# Autodesk Inventor assembly: Perna_Esq_Montada_v1
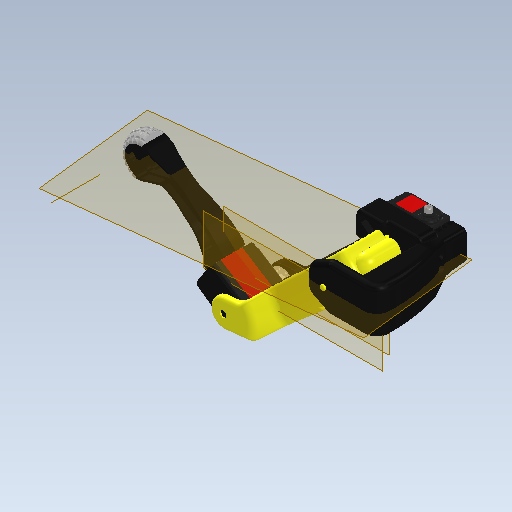
[picture p0: Inventor's stored thumbnail of the model, 512x512]
Saved by Autodesk Inventor 2020 (Build 240168000, 168)
## iProperties
Created: 2021-05-13
Part Number: Perna_Esq_Montada_v1
Document SubType Name: Assembly
Designer: JCarlos
Author: JCarlos
## Documents named in this file (10)
- C:\Users\candu\Google Drive\Doutorado_UTFPR\Projeto_1_SpotMicro\Projeto_3D\Robo_Montado_v3\Perna_Esq_Montada_v3.iam
- C:\Users\candu\Google Drive\Doutorado_UTFPR\Projeto_1_SpotMicro\Projeto_3D\Robo_Montado_v3\Braço_Esq.ipt
- C:\Users\candu\Google Drive\Doutorado_UTFPR\Projeto_1_SpotMicro\Projeto_3D\Robo_Montado_v3\Ante_Braço_Esq.ipt
- C:\Users\candu\Google Drive\Doutorado_UTFPR\Projeto_1_SpotMicro\Projeto_3D\Perna_Esq_Montada_v1\Design Accelerator\Rolamento1.iam
- C:\Users\candu\Google Drive\Doutorado_UTFPR\Projeto_1_SpotMicro\Projeto_3D\Robo_Montado_v3\foot.ipt
- C:\Users\candu\Google Drive\Doutorado_UTFPR\Projeto_1_SpotMicro\Projeto_3D\Robo_Montado_v3\Cover_Braço_Esq_v3.ipt
- C:\Users\candu\Google Drive\Doutorado_UTFPR\Projeto_1_SpotMicro\Projeto_3D\Robo_Montado_v3\LF20MG\Circle Rudder.ipt
- C:\Users\candu\Google Drive\Doutorado_UTFPR\Projeto_1_SpotMicro\Projeto_3D\Robo_Montado_v3\LF20MG\LF20MG.ipt
- C:\Users\candu\Google Drive\Doutorado_UTFPR\Projeto_1_SpotMicro\Projeto_3D\Robo_Montado_v3\Rótula_FrEsq_TrDir_v3.ipt
- C:\Users\candu\Google Drive\Doutorado_UTFPR\Projeto_1_SpotMicro\Projeto_3D\Robo_Montado_v3\Ombrera_Esq.ipt
## Components (11 placed, 9 different names)
1. LF20MG:3 — Coincidência:46, Coincidência:47, Coincidência:48, Coincidência:49, Coincidência:50
2. Braço_Esq:1 — Coincidência:8, Alinhamento:3, Coincidência:44, Coincidência:45, Coincidência:46, Coincidência:47, Coincidência:48, Coincidência:62, Tangente:2
3. Ante_Braço_Esq:1 — Coincidência:5, Alinhamento:1, Coincidência:7, Simetria:1, Coincidência:34, Coincidência:36, Coincidência:43, Coincidência:51, Coincidência:52, Coincidência:53
4. Cover_Braço_Esq_v3:1 — Coincidência:5, Alinhamento:1, Coincidência:7, Coincidência:8, Ângulo:1, Tangente:1, Coincidência:33, Alinhamento:2, Coincidência:64, Coincidência:65
5. Rolamento:1 [sub-assembly] — Coincidência:33, Alinhamento:2
6. LF20MG:2 — Coincidência:51, Coincidência:52, Coincidência:53, Coincidência:54, Coincidência:55
7. Circle Rudder:1 — Coincidência:34, Coincidência:36, Coincidência:43, Coincidência:49, Coincidência:50
8. foot:1 — Alinhamento:3, Coincidência:44, Coincidência:45
9. Rótula_FrEsq_TrDir_v3:1 — Coincidência:54, Coincidência:55, Ângulo:2, Coincidência:56, Coincidência:57, Coincidência:58, Ângulo:3, Alinhamento:4
10. LF20MG:4 — Coincidência:56, Coincidência:57, Coincidência:58, Coincidência:59, Coincidência:60, Coincidência:61
11. Ombrera_Esq:1 — Coincidência:59, Coincidência:60, Coincidência:61
## Relationships (39: Mate 29, Flush 4, Angle 3, Tangent 2, Symmetry 1)
- Coincidência:5 [Mate]: Ante_Braço_Esq:1 ↔ Cover_Braço_Esq_v3:1
- Alinhamento:1 [Flush]: Ante_Braço_Esq:1 ↔ Cover_Braço_Esq_v3:1
- Coincidência:7 [Mate]: Ante_Braço_Esq:1 ↔ Cover_Braço_Esq_v3:1
- Coincidência:8 [Mate] (1 mm): Braço_Esq:1 ↔ Cover_Braço_Esq_v3:1
- Ângulo:1 [Angle] (0 deg): Cover_Braço_Esq_v3:1
- Tangente:1: Cover_Braço_Esq_v3:1
- Simetria:1 [Symmetry]: Ante_Braço_Esq:1
- Coincidência:33 [Mate]: Cover_Braço_Esq_v3:1 ↔ Rolamento:1
- Alinhamento:2 [Flush]: Cover_Braço_Esq_v3:1 ↔ Rolamento:1
- Coincidência:34 [Mate]: Ante_Braço_Esq:1 ↔ Circle Rudder:1
- Coincidência:36 [Mate]: Ante_Braço_Esq:1 ↔ Circle Rudder:1
- Coincidência:43 [Mate]: Ante_Braço_Esq:1 ↔ Circle Rudder:1
- Alinhamento:3 [Flush]: Braço_Esq:1 ↔ foot:1
- Coincidência:44 [Mate]: Braço_Esq:1 ↔ foot:1
- Coincidência:45 [Mate]: Braço_Esq:1 ↔ foot:1
- Coincidência:46 [Mate]: LF20MG:3 ↔ Braço_Esq:1
- Coincidência:47 [Mate]: LF20MG:3 ↔ Braço_Esq:1
- Coincidência:48 [Mate]: LF20MG:3 ↔ Braço_Esq:1
- Coincidência:49 [Mate] (-46 mm): LF20MG:3 ↔ Circle Rudder:1
- Coincidência:50 [Mate]: LF20MG:3 ↔ Circle Rudder:1
- Coincidência:51 [Mate]: Ante_Braço_Esq:1 ↔ LF20MG:2
- Coincidência:52 [Mate]: Ante_Braço_Esq:1 ↔ LF20MG:2
- Coincidência:53 [Mate]: Ante_Braço_Esq:1 ↔ LF20MG:2
- Coincidência:54 [Mate]: LF20MG:2 ↔ Rótula_FrEsq_TrDir_v3:1
- Coincidência:55 [Mate] (3 mm): LF20MG:2 ↔ Rótula_FrEsq_TrDir_v3:1
- Ângulo:2 [Angle] (90 deg): Rótula_FrEsq_TrDir_v3:1
- Coincidência:56 [Mate]: Rótula_FrEsq_TrDir_v3:1 ↔ LF20MG:4
- Coincidência:57 [Mate]: Rótula_FrEsq_TrDir_v3:1 ↔ LF20MG:4
- Coincidência:58 [Mate]: Rótula_FrEsq_TrDir_v3:1 ↔ LF20MG:4
- Coincidência:59 [Mate]: LF20MG:4 ↔ Ombrera_Esq:1
- Coincidência:60 [Mate]: LF20MG:4 ↔ Ombrera_Esq:1
- Coincidência:61 [Mate] (0.5 mm): LF20MG:4 ↔ Ombrera_Esq:1
- Coincidência:62 [Mate]: Braço_Esq:1
- Coincidência:63 [Mate]
- Ângulo:3 [Angle] (90 deg): Rótula_FrEsq_TrDir_v3:1
- Tangente:2: Braço_Esq:1
- Alinhamento:4 [Flush]: Rótula_FrEsq_TrDir_v3:1
- Coincidência:64 [Mate]: Cover_Braço_Esq_v3:1
- Coincidência:65 [Mate] (200 mm): Cover_Braço_Esq_v3:1
